# Autodesk Inventor assembly: V4.0-trebuchet-assembled-instructions
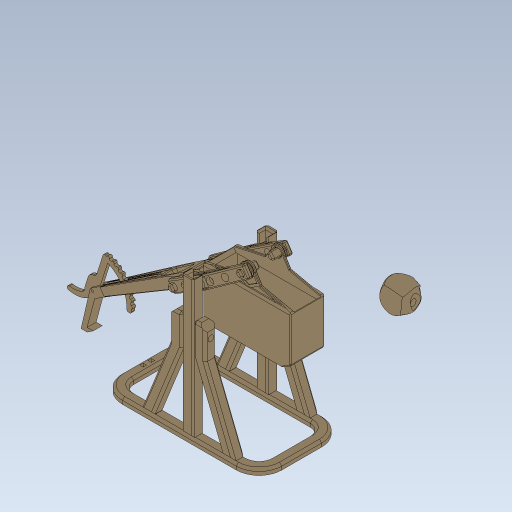
[picture p0: Inventor's stored thumbnail of the model, 512x512]
Saved by Autodesk Inventor 2023 (Build 270158030, 158C)
## iProperties
Created: 2024-12-20
Part Number: V4.0-trebuchet-assembled-instructions
Document SubType Name: Assembly
Designer: Imogen Heard
Author: Imogen Heard
## Documents named in this file (26)
- C:\Users\dheard\Documents\0004-inventor\3D-CAD-main\trebuchet\V4.0-trebuchet-assembled-instructions.iam
- C:\Users\dheard\Documents\0004-inventor\3D-CAD-main\trebuchet\pins.ipt
- C:\Users\dheard\Documents\0004-inventor\3D-CAD-main\trebuchet\bolder.ipt
- C:\Users\dheard\Documents\0004-inventor\3D-CAD-main\trebuchet\sling.ipt
- C:\Users\dheard\Documents\0004-inventor\3D-CAD-main\unicorn-horn\washers.ipt
- C:\Users\dheard\Documents\0004-inventor\3D-CAD-main\trebuchet\throw-ring.ipt
- C:\Users\dheard\Documents\0004-inventor\3D-CAD-main\trebuchet\border.ipt
- C:\Users\dheard\Documents\0004-inventor\3D-CAD-main\trebuchet\baseplate.ipt
- C:\Users\dheard\Documents\0004-inventor\3D-CAD-main\trebuchet\V4-upright-A.ipt
- C:\Users\dheard\Documents\0004-inventor\3D-CAD-main\trebuchet\V4-a-frame-A.ipt
- C:\Users\dheard\Documents\0004-inventor\3D-CAD-main\trebuchet\V4-pivot-A.ipt
- C:\Users\dheard\Documents\0004-inventor\3D-CAD-main\trebuchet\V4-throw-arm.ipt
- C:\Users\dheard\Documents\0004-inventor\3D-CAD-main\trebuchet\V4-ratchet.ipt
- C:\Users\dheard\Documents\0004-inventor\3D-CAD-main\trebuchet\V4-counterweight.ipt
- C:\Users\dheard\Documents\0004-inventor\3D-CAD-main\trebuchet\V4-pivot-B.ipt
- C:\Users\dheard\Documents\0004-inventor\3D-CAD-main\trebuchet\V4-upright-B.ipt
- C:\Users\dheard\Documents\0004-inventor\3D-CAD-main\trebuchet\V4-a-frame-B.ipt
- C:\Users\dheard\Documents\0004-inventor\3D-CAD-main\trebuchet\V4-a-frame-C.ipt
- C:\Users\dheard\Documents\0004-inventor\3D-CAD-main\trebuchet\V4-a-frame-D.ipt
- C:\Users\dheard\Documents\0004-inventor\3D-CAD-main\trebuchet\V4-spacer-A.ipt
- C:\Users\dheard\Documents\0004-inventor\3D-CAD-main\trebuchet\V4-spacer-B.ipt
- C:\Users\dheard\Documents\0004-inventor\3D-CAD-main\trebuchet\v4-latch.ipt
- C:\Users\dheard\Documents\0004-inventor\3D-CAD-main\trebuchet\V4-pegs.ipt
- C:\Users\dheard\Documents\0004-inventor\3D-CAD-main\trebuchet\V4.1-5x17mm-pin.ipt
- C:\Users\dheard\Documents\0004-inventor\3D-CAD-main\trebuchet\V4.1-6x16mm-pin.ipt
- C:\Users\dheard\Documents\0004-inventor\3D-CAD-main\trebuchet\V4.1-6x23mm-pin.ipt
## Components (33 placed, 25 different names)
1. pins:1 — Flush:7, Flush:25, Flush:26, Flush:27, Flush:28, Flush:29, Flush:30, Flush:31, Flush:32, Flush:33, Flush:34, Flush:35, Flush:36, Flush:37, Flush:38, Flush:39
2. bolder:1
3. sling:1 — Flush:40
4. washers:1 — Insert:9, Insert:10
5. washers:2 — Insert:11
6. throw-ring:1 — Flush:18
7. border:1 — Flush:7, Flush:18, Flush:25, Flush:26, Flush:27, Flush:28, Flush:29, Flush:30, Flush:31, Flush:32, Flush:33, Flush:34, Flush:35, Flush:36, Flush:37, Flush:38, Flush:39, Flush:40, Flush:42
8. V4-baseplate:1 — Flush:42, Flush:43, Angle:1
9. V4-upright-A:1 — Rotational:1
10. V4-a-frame-A:1 — Insert:16
11. V4-pivot-A:1 — Rotational:1, Insert:1, Insert:2, Insert:9, Insert:17, Insert:20, Insert:22
12. V4-throw-arm:1 — Insert:3, Insert:4, Insert:6, Insert:7, Insert:12
13. V4-ratchet:1 — Insert:12
14. V4-counterweight:1 — Insert:10, Angle:1
15. V4-pivot-B:1 — Insert:5, Insert:8, Insert:11, Insert:18, Insert:19, Insert:21
16. V4-upright-B:1
17. V4-a-frame-B:1 — Insert:15
18. V4-a-frame-C:1 — Insert:13
19. V4-a-frame-D:1 — Insert:14
20. V4-spacer-A:1 — Insert:1, Insert:2, Insert:3, Insert:4
21. V4-spacer-B:1 — Insert:5, Insert:6, Insert:7, Insert:8
22. v4-latch:1 — Flush:43, Flush:44
23. V4-pegs:1 — Flush:44
24. V4.1-5x17mm-pin:1 — Insert:13
25. V4.1-6x16mm-pin:1 — Insert:17
26. V4.1-6x23mm-pin:1 — Insert:22
27. V4.1-5x17mm-pin:2 — Insert:15
28. V4.1-5x17mm-pin:3 — Insert:16
29. V4.1-5x17mm-pin:4 — Insert:14
30. V4.1-6x16mm-pin:2 — Insert:18
31. V4.1-6x23mm-pin:2 — Insert:19
32. V4.1-6x23mm-pin:3 — Insert:21
33. V4.1-6x23mm-pin:4 — Insert:20
## Relationships (45: Insert 22, Flush 21, RevoluteJoint 1, Angle 1)
- Flush:7: pins:1 ↔ border:1
- Flush:18: throw-ring:1 ↔ border:1
- Flush:25: pins:1 ↔ border:1
- Flush:26: pins:1 ↔ border:1
- Flush:27: pins:1 ↔ border:1
- Flush:28: pins:1 ↔ border:1
- Flush:29: pins:1 ↔ border:1
- Flush:30: pins:1 ↔ border:1
- Flush:31: pins:1 ↔ border:1
- Flush:32: pins:1 ↔ border:1
- Flush:33: pins:1 ↔ border:1
- Flush:34: pins:1 ↔ border:1
- Flush:35: pins:1 ↔ border:1
- Flush:36: pins:1 ↔ border:1
- Flush:37: pins:1 ↔ border:1
- Flush:38: pins:1 ↔ border:1
- Flush:39: pins:1 ↔ border:1
- Flush:40: sling:1 ↔ border:1
- Flush:42: border:1 ↔ V4-baseplate:1
- Rotational:1 [RevoluteJoint] (-5.4 mm): V4-upright-A:1 ↔ V4-pivot-A:1
- Insert:1: V4-pivot-A:1 ↔ V4-spacer-A:1
- Insert:2: V4-pivot-A:1 ↔ V4-spacer-A:1
- Insert:3: V4-throw-arm:1 ↔ V4-spacer-A:1
- Insert:4: V4-throw-arm:1 ↔ V4-spacer-A:1
- Insert:5: V4-pivot-B:1 ↔ V4-spacer-B:1
- Insert:6: V4-throw-arm:1 ↔ V4-spacer-B:1
- Insert:7: V4-throw-arm:1 ↔ V4-spacer-B:1
- Insert:8: V4-pivot-B:1 ↔ V4-spacer-B:1
- Flush:43: V4-baseplate:1 ↔ v4-latch:1
- Flush:44: v4-latch:1 ↔ V4-pegs:1
- Insert:9: washers:1 ↔ V4-pivot-A:1
- Insert:10: washers:1 ↔ V4-counterweight:1
- Angle:1 (180 deg): V4-baseplate:1 ↔ V4-counterweight:1
- Insert:11: washers:2 ↔ V4-pivot-B:1
- Insert:12: V4-throw-arm:1 ↔ V4-ratchet:1
- Insert:13 (-13 mm): V4-a-frame-C:1 ↔ V4.1-5x17mm-pin:1
- Insert:14 (-3 mm): V4-a-frame-D:1 ↔ V4.1-5x17mm-pin:4
- Insert:15 (-13 mm): V4-a-frame-B:1 ↔ V4.1-5x17mm-pin:2
- Insert:16 (-13 mm): V4-a-frame-A:1 ↔ V4.1-5x17mm-pin:3
- Insert:17 (-5 mm): V4-pivot-A:1 ↔ V4.1-6x16mm-pin:1
- Insert:18 (-5 mm): V4-pivot-B:1 ↔ V4.1-6x16mm-pin:2
- Insert:19 (-7 mm): V4-pivot-B:1 ↔ V4.1-6x23mm-pin:2
- Insert:20 (-7 mm): V4-pivot-A:1 ↔ V4.1-6x23mm-pin:4
- Insert:21 (-7 mm): V4-pivot-B:1 ↔ V4.1-6x23mm-pin:3
- Insert:22 (-7 mm): V4-pivot-A:1 ↔ V4.1-6x23mm-pin:1
